# Autodesk Inventor assembly: Middle layer
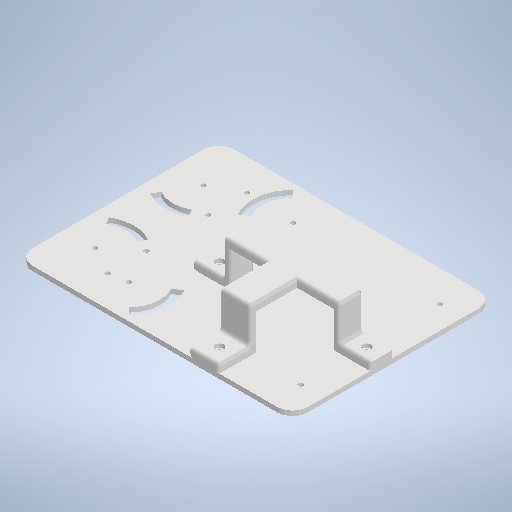
[picture p0: Inventor's stored thumbnail of the model, 512x512]
Saved by Autodesk Inventor 2025.1 (Build 291241000, 241)
## iProperties
Created: 2024-10-04
Part Number: Middle layer
Document SubType Name: Assembly
Designer: bw1293
Author: bw1293
## Documents named in this file (3)
- C:\Users\benja\OneDrive\Documents\PlatformIO\Projects\241025-214150-nano33ble\GEOFF-2.0\CAD\Middle layer.iam
- C:\Users\benja\OneDrive\Documents\PlatformIO\Projects\241025-214150-nano33ble\GEOFF-2.0\CAD\Middle layer.ipt
- C:\Users\benja\OneDrive\Documents\PlatformIO\Projects\241025-214150-nano33ble\GEOFF-2.0\CAD\Battery mount.ipt
## Components (2 placed, 2 different names)
1. Middle layer:1 — Insert:1
2. Battery mount:1 — Insert:1
## Relationships (1: Insert 1)
- Insert:1: Middle layer:1 ↔ Battery mount:1
